# Autodesk Inventor assembly: ASY GBK 1210 long wall shield 3
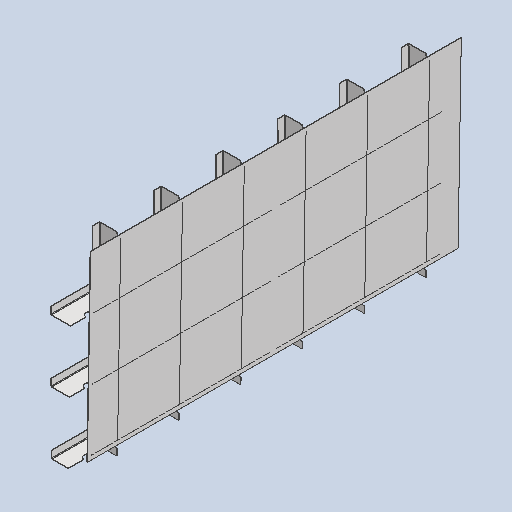
[picture p0: Inventor's stored thumbnail of the model, 512x512]
Saved by Autodesk Inventor 2026.2 (Build 302298000, 298)
## iProperties
Created: 2026-05-07
Part Number: ASY GBK 1210 long wall shield 3
Document SubType Name: Assembly
Designer: pokla
Mass: 252568 g
Surface Area: 163192 cm^2
Volume: 32174.3 cm^3
Density: 7.85 g/cm^3
Stock Number: 1211
Author: admin
## Documents named in this file (7)
- C:\Users\admin\Documents\Inventor\GBK-Gubkinskiy\ASY GBK 1210 long wall shield 3.iam
- C:\Users\admin\Documents\Inventor\GBK-Gubkinskiy\GBK 1018 shield 2.ipt
- C:\Users\admin\Documents\Inventor\GBK-Gubkinskiy\GBK 1211 second rib.ipt
- C:\Users\admin\Documents\Inventor\GBK-Gubkinskiy\0241 GBK stringer 4.ipt
- C:\Users\admin\Documents\Inventor\GBK-Gubkinskiy\0242 GBK stringer 5.ipt
- C:\Users\admin\Documents\Inventor\GBK-Gubkinskiy\0243 GBK stringer 6.ipt
- C:\Users\admin\Documents\Inventor\GBK-Gubkinskiy\GBK 1111 main rib.ipt
## Components (13 placed, 5 different names)
1. GBK 1212 stringer 4:1
2. GBK 1212 stringer 4:2
3. GBK 1213 stringer 5:1
4. GBK 1213 stringer 5:2
5. GBK 1214 stringer 6:1
6. GBK 1214 stringer 6:2
7. GBK 1018 shield 2:1
8. GBK 1211 second rib:1
9. GBK 1211 second rib:2
10. GBK 1211 second rib:3
11. GBK 1211 second rib:4
12. GBK 1211 second rib:5
13. GBK 1211 second rib:6
## Component patterns: (6 elements, first: GBK 1211 second rib:1)
## Relationships (9: WeldJoint 6, Mate 2, Flush 1)
- [Flush] (250 mm): GBK 1018 shield 2:1 ↔ GBK 1211 second rib:1
- [Mate]: GBK 1018 shield 2:1 ↔ GBK 1211 second rib:1
- [Mate]: GBK 1018 shield 2:1 ↔ GBK 1211 second rib:1
- [WeldJoint]: GBK 1212 stringer 4:1 ↔ GBK 1212 stringer 4:2
- [WeldJoint]: GBK 1213 stringer 5:1 ↔ GBK 1213 stringer 5:2
- [WeldJoint]: GBK 1214 stringer 6:1 ↔ GBK 1214 stringer 6:2
- [WeldJoint] (4 mm): GBK 1214 stringer 6:1 ↔ GBK 1211 second rib:1
- [WeldJoint] (4 mm): GBK 1213 stringer 5:1 ↔ GBK 1211 second rib:1
- [WeldJoint] (4 mm): GBK 1212 stringer 4:1 ↔ GBK 1211 second rib:1
## Named parameters: Шаг_шпангоутов = 496.66667 mm
